# Autodesk Inventor assembly: Box Arm
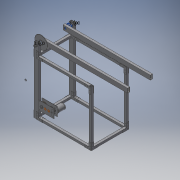
[picture p0: Inventor's stored thumbnail of the model, 180x180]
Saved by Autodesk Inventor 2018 (Build 220112000, 112)
## iProperties
Created: 2019-01-16
Part Number: Box Arm
Document SubType Name: Assembly
Designer: Gabriel
Author: Gabriel
## Documents named in this file (27)
- C:\Users\S-2513398\Downloads\2019CAD-master\2019CAD-master\Drivebase Box Arm\Box Arm.iam
- C:\Users\S-2513398\Downloads\2019CAD-master\2019CAD-master\Drivebase Box Arm\30in 1x1 Beam.ipt
- C:\Users\S-2513398\Downloads\2019CAD-master\2019CAD-master\Drivebase Box Arm\25in 1x1 Beam.ipt
- C:\Users\S-2513398\Downloads\2019CAD-master\2019CAD-master\Drivebase Box Arm\17in 1x1 Beam.ipt
- C:\Users\S-2513398\Downloads\2019CAD-master\2019CAD-master\Drivebase Box Arm\23in 1x1 Beam.ipt
- C:\Users\S-2513398\Downloads\2019CAD-master\2019CAD-master\Drivebase Box Arm\L gusset.ipt
- C:\Users\S-2513398\Downloads\2019CAD-master\2019CAD-master\Drivebase Box Arm\34.48in Arm Bea.ipt
- C:\Users\S-2513398\Downloads\2019CAD-master\2019CAD-master\Drivebase Box Arm\0_500_ID_x_1_125_OD_x_0_313_WD_Flanged_Bearing_217-2731.ipt
- C:\Users\S-2513398\Downloads\2019CAD-master\2019CAD-master\Drivebase Box Arm\_72t_Aluminum_Plate_Sprocket_25_Chain_1-1_8_Bearing_Bore_217-2627.ipt
- C:\Users\S-2513398\Downloads\2019CAD-master\2019CAD-master\Drivebase Box Arm\Hex Hub.ipt
- C:\Users\S-2513398\Downloads\2019CAD-master\2019CAD-master\Drivebase Box Arm\0.5in Hex Shaft.ipt
- C:\Users\S-2513398\Downloads\2019CAD-master\2019CAD-master\Drivebase Box Arm\1_2_Acetal_Spacer_-_1_2_Hex_217-3261.ipt
- C:\Users\S-2513398\Downloads\2019CAD-master\2019CAD-master\Drivebase Box Arm\am-0150 Toughbox Large Output Gear.ipt
- C:\Users\S-2513398\Downloads\2019CAD-master\2019CAD-master\Drivebase Box Arm\Mini_CIM_Motor_217-3371.ipt
- C:\Users\S-2513398\Downloads\2019CAD-master\2019CAD-master\Drivebase Box Arm\ARm Gearbox Plate.ipt
- C:\Users\S-2513398\Downloads\2019CAD-master\2019CAD-master\Drivebase Box Arm\1_16_Acetal_Spacer_-_1_2_Hex_217-3257.ipt
- C:\Users\S-2513398\Downloads\2019CAD-master\2019CAD-master\Drivebase Box Arm\3_8in Hex Shaft.ipt
- C:\Users\S-2513398\Downloads\2019CAD-master\2019CAD-master\Drivebase Box Arm\10T_Steel_Spur_Gear_20_DP_12T_Center_Distance_CIM_Motor_217-6334.ipt
- C:\Users\S-2513398\Downloads\2019CAD-master\2019CAD-master\Drivebase Box Arm\am-0143 50 Tooth 20 dp Aluminum Gear 375 Hex.ipt
- C:\Users\S-2513398\Downloads\2019CAD-master\2019CAD-master\Drivebase Box Arm\am-0151 14T 20dp 375hex.ipt
- C:\Users\S-2513398\Downloads\2019CAD-master\2019CAD-master\Drivebase Box Arm\1_16_Acetal_Spacer_-_3_8_Hex_217-3258.ipt
- C:\Users\S-2513398\Downloads\2019CAD-master\2019CAD-master\Drivebase Box Arm\40t_Aluminum_Spur_Gear_20_DP_3_8_Hex_Bore_217-2707.ipt
- C:\Users\S-2513398\Downloads\2019CAD-master\2019CAD-master\Drivebase Box Arm\am-0028 00.375'' id Flanged, Shielded Ball Bearing (FR6ZZ).ipt
- C:\Users\S-2513398\Downloads\2019CAD-master\2019CAD-master\Drivebase Box Arm\92196A271_18-8 STAINLESS STEEL SOCKET HEAD CAP SCREW.ipt
- C:\Users\S-2513398\Downloads\2019CAD-master\2019CAD-master\Drivebase Box Arm\am-3621 - S25-18HA-500H.ipt
- C:\Users\S-2513398\Downloads\2019CAD-master\2019CAD-master\Drivebase Box Arm\Clamping_Shaft_Collar_-_1_2_Hex_ID_217-2737.ipt
- C:\Users\S-2513398\Downloads\#10 Washer.ipt
## Components (89 placed, 26 different names)
1. 30in 1x1 Beam:1 — Mate:13, Mate:14, Mate:37, Mate:38, Mate:74, Mate:75, Mate:83, Mate:84, Mate:98, Mate:99, Mate:101, Mate:102, Mate:103, Mate:104
2. 30in 1x1 Beam:2 — Mate:11, Mate:12, Mate:39, Mate:40, Mate:73, Mate:76, Mate:86, Mate:87, Mate:95, Mate:96, Mate:105, Mate:106, Mate:107, Mate:108, Mate:441, Mate:442
3. 25in 1x1 Beam:1 — Mate:57, Mate:58, Mate:59, Mate:60, Mate:65, Mate:66, Mate:90, Mate:91
4. 25in 1x1 Beam:2 — Mate:61, Mate:62, Mate:63, Mate:64, Mate:67, Mate:68, Mate:93, Mate:94
5. 25in 1x1 Beam:3 — Mate:29, Mate:30, Mate:53, Mate:54, Mate:97, Mate:443
6. 25in 1x1 Beam:4 — Mate:31, Mate:32, Mate:55, Mate:56, Mate:100
7. 17in 1x1 Beam:1 — Mate:69, Mate:70, Mate:71, Mate:72
8. 17in 1x1 Beam:2 — Mate:21, Mate:22, Mate:23, Mate:24
9. 23in 1x1 Beam:1 — Mate:43, Mate:44, Mate:49, Mate:50, Mate:88, Mate:92
10. 23in 1x1 Beam:2 — Mate:47, Mate:48, Mate:51, Mate:52, Mate:85, Mate:89
11. L gusset:1 — Mate:53, Mate:54, Mate:63, Mate:64
12. L gusset:4 — Mate:49, Mate:50, Mate:61, Mate:62
13. L gusset:5 — Mate:51, Mate:52, Mate:57, Mate:58
14. L gusset:7 — Mate:11, Mate:12, Mate:23, Mate:24
15. L gusset:9 — Mate:13, Mate:14, Mate:21, Mate:22
16. L gusset:11 — Mate:31, Mate:32, Mate:74, Mate:75
17. L gusset:12 — Mate:29, Mate:30, Mate:73, Mate:76
18. L gusset:13 — Mate:43, Mate:44
19. L gusset:14 — Mate:47, Mate:48
20. L gusset:15 — Mate:39, Mate:40, Mate:77, Mate:80
21. L gusset:16 — Mate:37, Mate:38, Mate:78, Mate:79
22. L gusset:17 — Mate:55, Mate:56, Mate:59, Mate:60
23. L gusset:18 — Mate:67, Mate:68, Mate:69, Mate:70
24. L gusset:19 — Mate:65, Mate:66, Mate:71, Mate:72
25. 17in 1x1 Beam:3 — Mate:77, Mate:78, Mate:79, Mate:80
26. 34.48in Arm Bea:2 — Mate:109, Mate:110
27. 0_500_ID_x_1_125_OD_x_0_313_WD_Flanged_Bearing_217-2731:1 — Mate:103, Mate:104, Mate:139, Mate:140, Mate:149
28. 0_500_ID_x_1_125_OD_x_0_313_WD_Flanged_Bearing_217-2731:2 — Mate:107, Mate:108, Mate:126, Mate:152
29. 0_500_ID_x_1_125_OD_x_0_313_WD_Flanged_Bearing_217-2731:5 — Mate:101, Mate:102, Mate:143
30. 0_500_ID_x_1_125_OD_x_0_313_WD_Flanged_Bearing_217-2731:8 — Mate:105, Mate:106, Mate:446, Mate:447
31. L gusset:20 — Mate:92, Mate:93, Mate:94
32. L gusset:21 — Mate:89, Mate:90, Mate:91
33. L gusset:22 — Mate:98, Mate:99, Mate:100
34. L gusset:23 — Mate:95, Mate:96, Mate:97
35. L gusset:24 — Mate:83, Mate:84, Mate:85
36. L gusset:25 — Mate:86, Mate:87, Mate:88
37. _72t_Aluminum_Plate_Sprocket_25_Chain_1-1_8_Bearing_Bore_217-2627:2 — Mate:120, Mate:121, Mate:138, Flush:4
38. Hex Hub:2 — Mate:109, Mate:110, Mate:111, Mate:112, Mate:113
39. Hex Hub:3 — Mate:120, Mate:121, Mate:138, Mate:444, Mate:445
40. 1_2_Acetal_Spacer_-_1_2_Hex_217-3261:1 — Mate:126, Mate:406
41. 1_2_Acetal_Spacer_-_1_2_Hex_217-3261:3 — Mate:111, Mate:112, Mate:113
42. 34.48in Arm Bea:3 — Mate:128
43. Hex Hub:4 — Mate:136, Mate:139, Mate:140
44. Hex Hub:5 — Mate:128, Mate:133
45. 1_2_Acetal_Spacer_-_1_2_Hex_217-3261:7 — Mate:143, Mate:403
46. 1_2_Acetal_Spacer_-_1_2_Hex_217-3261:8 — Mate:133, Mate:136
47. 1_2_Acetal_Spacer_-_1_2_Hex_217-3261:9 — Mate:149
48. 1_2_Acetal_Spacer_-_1_2_Hex_217-3261:10 — Mate:152
49. 0.5in Hex Shaft:5 — Mate:345, Mate:346, Mate:347, Mate:348, Mate:349, Mate:350, Mate:351, Mate:386, Mate:387, Mate:389, Mate:390, Mate:395, Mate:396, Mate:398, Mate:399, Rotation:1, Mate:437, Mate:438, Flush:3
50. Mini_CIM_Motor_217-3371:5 — Mate:431, Mate:432, Mate:433, Mate:434, Mate:435, Mate:436
51. am-0150 Toughbox Large Output Gear:8 — Mate:345, Mate:346, Mate:347, Mate:352
52. 1_16_Acetal_Spacer_-_1_2_Hex_217-3257:4 — Mate:348, Mate:349, Mate:352, Mate:353
53. 1_16_Acetal_Spacer_-_1_2_Hex_217-3257:6 — Mate:350, Mate:351, Mate:353, Mate:354
54. 3_8in Hex Shaft:5 — Mate:313, Mate:314, Mate:315, Mate:316, Mate:317, Mate:318, Mate:321, Mate:322, Mate:357, Mate:358, Mate:411, Flush:2, Mate:425, Rotation:2
55. am-0151 14T 20dp 375hex:1 — Mate:325, Mate:326, Mate:331, Mate:335
56. am-0151 14T 20dp 375hex:3 — Mate:315, Mate:316, Mate:320, Mate:359
57. am-0143 50 Tooth 20 dp Aluminum Gear 375 Hex:5 — Mate:327, Mate:328, Mate:332, Mate:339
58. 10T_Steel_Spur_Gear_20_DP_12T_Center_Distance_CIM_Motor_217-6334:6 — Mate:434, Mate:435, Mate:436
59. 1_16_Acetal_Spacer_-_3_8_Hex_217-3258:2 — Mate:337, Mate:338, Mate:339
60. 1_16_Acetal_Spacer_-_3_8_Hex_217-3258:3 — Mate:333, Mate:334, Mate:335, Mate:422
61. 1_16_Acetal_Spacer_-_3_8_Hex_217-3258:5 — Mate:321, Mate:322, Mate:323, Mate:423
62. 1_16_Acetal_Spacer_-_3_8_Hex_217-3258:6 — Mate:317, Mate:318, Mate:319, Mate:320
63. 40t_Aluminum_Spur_Gear_20_DP_3_8_Hex_Bore_217-2707:1 — Mate:313, Mate:314, Mate:319, Mate:323
64. 3_8in Hex Shaft:10 — Mate:325, Mate:326, Mate:327, Mate:328, Mate:329, Mate:330, Mate:333, Mate:334, Mate:337, Mate:338, Mate:412, Flush:1, Mate:424, Mate:426, Rotation:3
65. ARm Gearbox Plate:5 — Mate:341, Mate:344, Mate:413, Mate:414, Mate:415, Mate:416, Mate:441, Mate:442, Mate:443
66. ARm Gearbox Plate:6 — Mate:342, Mate:343, Mate:360, Mate:361, Mate:362, Mate:363, Mate:407, Mate:408, Mate:409, Mate:410, Mate:419, Mate:421, Rotation:1
67. 1_16_Acetal_Spacer_-_3_8_Hex_217-3258:8 — Mate:357, Mate:358, Mate:359
68. 1_16_Acetal_Spacer_-_3_8_Hex_217-3258:10 — Mate:329, Mate:330, Mate:331, Mate:332
69. 0_500_ID_x_1_125_OD_x_0_313_WD_Flanged_Bearing_217-2731:9 — Mate:341, Mate:344, Mate:439
70. 0_500_ID_x_1_125_OD_x_0_313_WD_Flanged_Bearing_217-2731:10 — Mate:342, Mate:343, Mate:354
71. 92196A271_18-8 STAINLESS STEEL SOCKET HEAD CAP SCREW:1 — Mate:361, Mate:363, Mate:420, Mate:429, Mate:431
72. 92196A271_18-8 STAINLESS STEEL SOCKET HEAD CAP SCREW:2 — Mate:360, Mate:362, Mate:417, Mate:427, Mate:432
73. am-0028 00.375'' id Flanged, Shielded Ball Bearing (FR6ZZ):3 — Mate:414, Mate:416, Mate:425, Rotation:2
74. am-0028 00.375'' id Flanged, Shielded Ball Bearing (FR6ZZ):4 — Mate:413, Mate:415, Mate:424, Mate:426, Rotation:3
75. am-3621 - S25-18HA-500H:1 — Mate:386, Mate:387, Flush:4
76. 1_2_Acetal_Spacer_-_1_2_Hex_217-3261:11 — Mate:389, Mate:390, Mate:397
77. Clamping_Shaft_Collar_-_1_2_Hex_ID_217-2737:1 — Mate:395, Mate:396, Mate:397, Flush:3
78. Clamping_Shaft_Collar_-_1_2_Hex_ID_217-2737:2 — Mate:398, Mate:399, Mate:440
79. Clamping_Shaft_Collar_-_1_2_Hex_ID_217-2737:5 — Mate:406
80. Clamping_Shaft_Collar_-_1_2_Hex_ID_217-2737:6 — Mate:403
81. am-0028 00.375'' id Flanged, Shielded Ball Bearing (FR6ZZ):5 — Mate:409, Mate:410, Mate:411, Flush:2, Mate:423
82. am-0028 00.375'' id Flanged, Shielded Ball Bearing (FR6ZZ):6 — Mate:407, Mate:408, Mate:412, Flush:1, Mate:422
83. #10 Washer:1 — Mate:417, Mate:419, Mate:428
84. #10 Washer:2 — Mate:420, Mate:421, Mate:430
85. #10 Washer:3 — Mate:427, Mate:428, Mate:433
86. #10 Washer:4 — Mate:429, Mate:430
87. 1_16_Acetal_Spacer_-_1_2_Hex_217-3257:9 — Mate:437, Mate:438, Mate:439, Mate:440
88. 1_16_Acetal_Spacer_-_1_2_Hex_217-3257:10
89. 1_2_Acetal_Spacer_-_1_2_Hex_217-3261:12 — Mate:444, Mate:445, Mate:446, Mate:447
## Relationships (199: Mate 192, Flush 4, RelateRotation 3)
- Mate:11: 30in 1x1 Beam:2 ↔ L gusset:7
- Mate:12: 30in 1x1 Beam:2 ↔ L gusset:7
- Mate:13: 30in 1x1 Beam:1 ↔ L gusset:9
- Mate:14: 30in 1x1 Beam:1 ↔ L gusset:9
- Mate:21: 17in 1x1 Beam:2 ↔ L gusset:9
- Mate:22: 17in 1x1 Beam:2 ↔ L gusset:9
- Mate:23: 17in 1x1 Beam:2 ↔ L gusset:7
- Mate:24: 17in 1x1 Beam:2 ↔ L gusset:7
- Mate:29: 25in 1x1 Beam:3 ↔ L gusset:12
- Mate:30: 25in 1x1 Beam:3 ↔ L gusset:12
- Mate:31: 25in 1x1 Beam:4 ↔ L gusset:11
- Mate:32: 25in 1x1 Beam:4 ↔ L gusset:11
- Mate:37: 30in 1x1 Beam:1 ↔ L gusset:16
- Mate:38: 30in 1x1 Beam:1 ↔ L gusset:16
- Mate:39: 30in 1x1 Beam:2 ↔ L gusset:15
- Mate:40: 30in 1x1 Beam:2 ↔ L gusset:15
- Mate:43: 23in 1x1 Beam:1 ↔ L gusset:13
- Mate:44: 23in 1x1 Beam:1 ↔ L gusset:13
- Mate:47: 23in 1x1 Beam:2 ↔ L gusset:14
- Mate:48: 23in 1x1 Beam:2 ↔ L gusset:14
- Mate:49: 23in 1x1 Beam:1 ↔ L gusset:4
- Mate:50: 23in 1x1 Beam:1 ↔ L gusset:4
- Mate:51: 23in 1x1 Beam:2 ↔ L gusset:5
- Mate:52: 23in 1x1 Beam:2 ↔ L gusset:5
- Mate:53: 25in 1x1 Beam:3 ↔ L gusset:1
- Mate:54: 25in 1x1 Beam:3 ↔ L gusset:1
- Mate:55: 25in 1x1 Beam:4 ↔ L gusset:17
- Mate:56: 25in 1x1 Beam:4 ↔ L gusset:17
- Mate:57: 25in 1x1 Beam:1 ↔ L gusset:5
- Mate:58: 25in 1x1 Beam:1 ↔ L gusset:5
- Mate:59: 25in 1x1 Beam:1 ↔ L gusset:17
- Mate:60: 25in 1x1 Beam:1 ↔ L gusset:17
- Mate:61: 25in 1x1 Beam:2 ↔ L gusset:4
- Mate:62: 25in 1x1 Beam:2 ↔ L gusset:4
- Mate:63: 25in 1x1 Beam:2 ↔ L gusset:1
- Mate:64: 25in 1x1 Beam:2 ↔ L gusset:1
- Mate:65: 25in 1x1 Beam:1 ↔ L gusset:19
- Mate:66: 25in 1x1 Beam:1 ↔ L gusset:19
- Mate:67: 25in 1x1 Beam:2 ↔ L gusset:18
- Mate:68: 25in 1x1 Beam:2 ↔ L gusset:18
- Mate:69: 17in 1x1 Beam:1 ↔ L gusset:18
- Mate:70: 17in 1x1 Beam:1 ↔ L gusset:18
- Mate:71: 17in 1x1 Beam:1 ↔ L gusset:19
- Mate:72: 17in 1x1 Beam:1 ↔ L gusset:19
- Mate:73: 30in 1x1 Beam:2 ↔ L gusset:12
- Mate:74: 30in 1x1 Beam:1 ↔ L gusset:11
- Mate:75: 30in 1x1 Beam:1 ↔ L gusset:11
- Mate:76: 30in 1x1 Beam:2 ↔ L gusset:12
- Mate:77: L gusset:15 ↔ 17in 1x1 Beam:3
- Mate:78: L gusset:16 ↔ 17in 1x1 Beam:3
- Mate:79: L gusset:16 ↔ 17in 1x1 Beam:3
- Mate:80: L gusset:15 ↔ 17in 1x1 Beam:3
- Mate:83: 30in 1x1 Beam:1 ↔ L gusset:24
- Mate:84: 30in 1x1 Beam:1 ↔ L gusset:24
- Mate:85: 23in 1x1 Beam:2 ↔ L gusset:24
- Mate:86: 30in 1x1 Beam:2 ↔ L gusset:25
- Mate:87: 30in 1x1 Beam:2 ↔ L gusset:25
- Mate:88: 23in 1x1 Beam:1 ↔ L gusset:25
- Mate:89: 23in 1x1 Beam:2 ↔ L gusset:21
- Mate:90: 25in 1x1 Beam:1 ↔ L gusset:21
- Mate:91: 25in 1x1 Beam:1 ↔ L gusset:21
- Mate:92: 23in 1x1 Beam:1 ↔ L gusset:20
- Mate:93: 25in 1x1 Beam:2 ↔ L gusset:20
- Mate:94: 25in 1x1 Beam:2 ↔ L gusset:20
- Mate:95: 30in 1x1 Beam:2 ↔ L gusset:23
- Mate:96: 30in 1x1 Beam:2 ↔ L gusset:23
- Mate:97: 25in 1x1 Beam:3 ↔ L gusset:23
- Mate:98: 30in 1x1 Beam:1 ↔ L gusset:22
- Mate:99: 30in 1x1 Beam:1 ↔ L gusset:22
- Mate:100: 25in 1x1 Beam:4 ↔ L gusset:22
- Mate:101: 30in 1x1 Beam:1 ↔ 0_500_ID_x_1_125_OD_x_0_313_WD_Flanged_Bearing_217-2731:5
- Mate:102: 30in 1x1 Beam:1 ↔ 0_500_ID_x_1_125_OD_x_0_313_WD_Flanged_Bearing_217-2731:5
- Mate:103: 30in 1x1 Beam:1 ↔ 0_500_ID_x_1_125_OD_x_0_313_WD_Flanged_Bearing_217-2731:1
- Mate:104: 30in 1x1 Beam:1 ↔ 0_500_ID_x_1_125_OD_x_0_313_WD_Flanged_Bearing_217-2731:1
- Mate:105: 30in 1x1 Beam:2 ↔ 0_500_ID_x_1_125_OD_x_0_313_WD_Flanged_Bearing_217-2731:8
- Mate:106: 30in 1x1 Beam:2 ↔ 0_500_ID_x_1_125_OD_x_0_313_WD_Flanged_Bearing_217-2731:8
- Mate:107: 30in 1x1 Beam:2 ↔ 0_500_ID_x_1_125_OD_x_0_313_WD_Flanged_Bearing_217-2731:2
- Mate:108: 30in 1x1 Beam:2 ↔ 0_500_ID_x_1_125_OD_x_0_313_WD_Flanged_Bearing_217-2731:2
- Mate:109: 34.48in Arm Bea:2 ↔ Hex Hub:2
- Mate:110: 34.48in Arm Bea:2 ↔ Hex Hub:2
- Mate:111: Hex Hub:2 ↔ 1_2_Acetal_Spacer_-_1_2_Hex_217-3261:3
- Mate:112: Hex Hub:2 ↔ 1_2_Acetal_Spacer_-_1_2_Hex_217-3261:3
- Mate:113: Hex Hub:2 ↔ 1_2_Acetal_Spacer_-_1_2_Hex_217-3261:3
- Mate:120: _72t_Aluminum_Plate_Sprocket_25_Chain_1-1_8_Bearing_Bore_217-2627:2 ↔ Hex Hub:3
- Mate:121: _72t_Aluminum_Plate_Sprocket_25_Chain_1-1_8_Bearing_Bore_217-2627:2 ↔ Hex Hub:3
- Mate:126: 0_500_ID_x_1_125_OD_x_0_313_WD_Flanged_Bearing_217-2731:2 ↔ 1_2_Acetal_Spacer_-_1_2_Hex_217-3261:1
- Mate:128: 34.48in Arm Bea:3 ↔ Hex Hub:5
- Mate:133: Hex Hub:5 ↔ 1_2_Acetal_Spacer_-_1_2_Hex_217-3261:8
- Mate:136: Hex Hub:4 ↔ 1_2_Acetal_Spacer_-_1_2_Hex_217-3261:8
- Mate:138: _72t_Aluminum_Plate_Sprocket_25_Chain_1-1_8_Bearing_Bore_217-2627:2 ↔ Hex Hub:3
- Mate:139: 0_500_ID_x_1_125_OD_x_0_313_WD_Flanged_Bearing_217-2731:1 ↔ Hex Hub:4
- Mate:140: 0_500_ID_x_1_125_OD_x_0_313_WD_Flanged_Bearing_217-2731:1 ↔ Hex Hub:4
- Mate:143: 0_500_ID_x_1_125_OD_x_0_313_WD_Flanged_Bearing_217-2731:5 ↔ 1_2_Acetal_Spacer_-_1_2_Hex_217-3261:7
- Mate:149: 0_500_ID_x_1_125_OD_x_0_313_WD_Flanged_Bearing_217-2731:1 ↔ 1_2_Acetal_Spacer_-_1_2_Hex_217-3261:9
- Mate:152: 0_500_ID_x_1_125_OD_x_0_313_WD_Flanged_Bearing_217-2731:2 ↔ 1_2_Acetal_Spacer_-_1_2_Hex_217-3261:10
- Mate:313: 3_8in Hex Shaft:5 ↔ 40t_Aluminum_Spur_Gear_20_DP_3_8_Hex_Bore_217-2707:1
- Mate:314: 3_8in Hex Shaft:5 ↔ 40t_Aluminum_Spur_Gear_20_DP_3_8_Hex_Bore_217-2707:1
- Mate:315: 3_8in Hex Shaft:5 ↔ am-0151 14T 20dp 375hex:3
- Mate:316: 3_8in Hex Shaft:5 ↔ am-0151 14T 20dp 375hex:3
- Mate:317: 3_8in Hex Shaft:5 ↔ 1_16_Acetal_Spacer_-_3_8_Hex_217-3258:6
- Mate:318: 3_8in Hex Shaft:5 ↔ 1_16_Acetal_Spacer_-_3_8_Hex_217-3258:6
- Mate:319: 1_16_Acetal_Spacer_-_3_8_Hex_217-3258:6 ↔ 40t_Aluminum_Spur_Gear_20_DP_3_8_Hex_Bore_217-2707:1
- Mate:320: am-0151 14T 20dp 375hex:3 ↔ 1_16_Acetal_Spacer_-_3_8_Hex_217-3258:6
- Mate:321: 3_8in Hex Shaft:5 ↔ 1_16_Acetal_Spacer_-_3_8_Hex_217-3258:5
- Mate:322: 3_8in Hex Shaft:5 ↔ 1_16_Acetal_Spacer_-_3_8_Hex_217-3258:5
- Mate:323: 1_16_Acetal_Spacer_-_3_8_Hex_217-3258:5 ↔ 40t_Aluminum_Spur_Gear_20_DP_3_8_Hex_Bore_217-2707:1
- Mate:325: am-0151 14T 20dp 375hex:1 ↔ 3_8in Hex Shaft:10
- Mate:326: am-0151 14T 20dp 375hex:1 ↔ 3_8in Hex Shaft:10
- Mate:327: am-0143 50 Tooth 20 dp Aluminum Gear 375 Hex:5 ↔ 3_8in Hex Shaft:10
- Mate:328: am-0143 50 Tooth 20 dp Aluminum Gear 375 Hex:5 ↔ 3_8in Hex Shaft:10
- Mate:329: 3_8in Hex Shaft:10 ↔ 1_16_Acetal_Spacer_-_3_8_Hex_217-3258:10
- Mate:330: 3_8in Hex Shaft:10 ↔ 1_16_Acetal_Spacer_-_3_8_Hex_217-3258:10
- Mate:331: am-0151 14T 20dp 375hex:1 ↔ 1_16_Acetal_Spacer_-_3_8_Hex_217-3258:10
- Mate:332: am-0143 50 Tooth 20 dp Aluminum Gear 375 Hex:5 ↔ 1_16_Acetal_Spacer_-_3_8_Hex_217-3258:10
- Mate:333: 1_16_Acetal_Spacer_-_3_8_Hex_217-3258:3 ↔ 3_8in Hex Shaft:10
- Mate:334: 1_16_Acetal_Spacer_-_3_8_Hex_217-3258:3 ↔ 3_8in Hex Shaft:10
- Mate:335: am-0151 14T 20dp 375hex:1 ↔ 1_16_Acetal_Spacer_-_3_8_Hex_217-3258:3
- Mate:337: 1_16_Acetal_Spacer_-_3_8_Hex_217-3258:2 ↔ 3_8in Hex Shaft:10
- Mate:338: 1_16_Acetal_Spacer_-_3_8_Hex_217-3258:2 ↔ 3_8in Hex Shaft:10
- Mate:339: am-0143 50 Tooth 20 dp Aluminum Gear 375 Hex:5 ↔ 1_16_Acetal_Spacer_-_3_8_Hex_217-3258:2
- Mate:341: ARm Gearbox Plate:5 ↔ 0_500_ID_x_1_125_OD_x_0_313_WD_Flanged_Bearing_217-2731:9
- Mate:342: ARm Gearbox Plate:6 ↔ 0_500_ID_x_1_125_OD_x_0_313_WD_Flanged_Bearing_217-2731:10
- Mate:343: ARm Gearbox Plate:6 ↔ 0_500_ID_x_1_125_OD_x_0_313_WD_Flanged_Bearing_217-2731:10
- Mate:344: ARm Gearbox Plate:5 ↔ 0_500_ID_x_1_125_OD_x_0_313_WD_Flanged_Bearing_217-2731:9
- Mate:345: 0.5in Hex Shaft:5 ↔ am-0150 Toughbox Large Output Gear:8
- Mate:346: 0.5in Hex Shaft:5 ↔ am-0150 Toughbox Large Output Gear:8
- Mate:347: 0.5in Hex Shaft:5 ↔ am-0150 Toughbox Large Output Gear:8
- Mate:348: 0.5in Hex Shaft:5 ↔ 1_16_Acetal_Spacer_-_1_2_Hex_217-3257:4
- Mate:349: 0.5in Hex Shaft:5 ↔ 1_16_Acetal_Spacer_-_1_2_Hex_217-3257:4
- Mate:350: 0.5in Hex Shaft:5 ↔ 1_16_Acetal_Spacer_-_1_2_Hex_217-3257:6
- Mate:351: 0.5in Hex Shaft:5 ↔ 1_16_Acetal_Spacer_-_1_2_Hex_217-3257:6
- Mate:352: am-0150 Toughbox Large Output Gear:8 ↔ 1_16_Acetal_Spacer_-_1_2_Hex_217-3257:4
- Mate:353: 1_16_Acetal_Spacer_-_1_2_Hex_217-3257:4 ↔ 1_16_Acetal_Spacer_-_1_2_Hex_217-3257:6
- Mate:354: 1_16_Acetal_Spacer_-_1_2_Hex_217-3257:6 ↔ 0_500_ID_x_1_125_OD_x_0_313_WD_Flanged_Bearing_217-2731:10
- Mate:357: 3_8in Hex Shaft:5 ↔ 1_16_Acetal_Spacer_-_3_8_Hex_217-3258:8
- Mate:358: 3_8in Hex Shaft:5 ↔ 1_16_Acetal_Spacer_-_3_8_Hex_217-3258:8
- Mate:359: am-0151 14T 20dp 375hex:3 ↔ 1_16_Acetal_Spacer_-_3_8_Hex_217-3258:8
- Mate:360: ARm Gearbox Plate:6 ↔ 92196A271_18-8 STAINLESS STEEL SOCKET HEAD CAP SCREW:2
- Mate:361: ARm Gearbox Plate:6 ↔ 92196A271_18-8 STAINLESS STEEL SOCKET HEAD CAP SCREW:1
- Mate:362: ARm Gearbox Plate:6 ↔ 92196A271_18-8 STAINLESS STEEL SOCKET HEAD CAP SCREW:2
- Mate:363: ARm Gearbox Plate:6 ↔ 92196A271_18-8 STAINLESS STEEL SOCKET HEAD CAP SCREW:1
- Mate:386: 0.5in Hex Shaft:5 ↔ am-3621 - S25-18HA-500H:1
- Mate:387: 0.5in Hex Shaft:5 ↔ am-3621 - S25-18HA-500H:1
- Mate:389: 0.5in Hex Shaft:5 ↔ 1_2_Acetal_Spacer_-_1_2_Hex_217-3261:11
- Mate:390: 0.5in Hex Shaft:5 ↔ 1_2_Acetal_Spacer_-_1_2_Hex_217-3261:11
- Mate:395: 0.5in Hex Shaft:5 ↔ Clamping_Shaft_Collar_-_1_2_Hex_ID_217-2737:1
- Mate:396: 0.5in Hex Shaft:5 ↔ Clamping_Shaft_Collar_-_1_2_Hex_ID_217-2737:1
- Mate:397: 1_2_Acetal_Spacer_-_1_2_Hex_217-3261:11 ↔ Clamping_Shaft_Collar_-_1_2_Hex_ID_217-2737:1
- Mate:398: 0.5in Hex Shaft:5 ↔ Clamping_Shaft_Collar_-_1_2_Hex_ID_217-2737:2
- Mate:399: 0.5in Hex Shaft:5 ↔ Clamping_Shaft_Collar_-_1_2_Hex_ID_217-2737:2
- Mate:403: 1_2_Acetal_Spacer_-_1_2_Hex_217-3261:7 ↔ Clamping_Shaft_Collar_-_1_2_Hex_ID_217-2737:6
- Mate:406: 1_2_Acetal_Spacer_-_1_2_Hex_217-3261:1 ↔ Clamping_Shaft_Collar_-_1_2_Hex_ID_217-2737:5
- Mate:407: ARm Gearbox Plate:6 ↔ am-0028 00.375'' id Flanged, Shielded Ball Bearing (FR6ZZ):6
- Mate:408: ARm Gearbox Plate:6 ↔ am-0028 00.375'' id Flanged, Shielded Ball Bearing (FR6ZZ):6
- Mate:409: ARm Gearbox Plate:6 ↔ am-0028 00.375'' id Flanged, Shielded Ball Bearing (FR6ZZ):5
- Mate:410: ARm Gearbox Plate:6 ↔ am-0028 00.375'' id Flanged, Shielded Ball Bearing (FR6ZZ):5
- Mate:411: 3_8in Hex Shaft:5 ↔ am-0028 00.375'' id Flanged, Shielded Ball Bearing (FR6ZZ):5
- Mate:412: 3_8in Hex Shaft:10 ↔ am-0028 00.375'' id Flanged, Shielded Ball Bearing (FR6ZZ):6
- Mate:413: ARm Gearbox Plate:5 ↔ am-0028 00.375'' id Flanged, Shielded Ball Bearing (FR6ZZ):4
- Mate:414: ARm Gearbox Plate:5 ↔ am-0028 00.375'' id Flanged, Shielded Ball Bearing (FR6ZZ):3
- Mate:415: ARm Gearbox Plate:5 ↔ am-0028 00.375'' id Flanged, Shielded Ball Bearing (FR6ZZ):4
- Mate:416: ARm Gearbox Plate:5 ↔ am-0028 00.375'' id Flanged, Shielded Ball Bearing (FR6ZZ):3
- Mate:417: 92196A271_18-8 STAINLESS STEEL SOCKET HEAD CAP SCREW:2 ↔ #10 Washer:1
- Mate:419: ARm Gearbox Plate:6 ↔ #10 Washer:1
- Mate:420: 92196A271_18-8 STAINLESS STEEL SOCKET HEAD CAP SCREW:1 ↔ #10 Washer:2
- Mate:421: ARm Gearbox Plate:6 ↔ #10 Washer:2
- Flush:1: 3_8in Hex Shaft:10 ↔ am-0028 00.375'' id Flanged, Shielded Ball Bearing (FR6ZZ):6
- Flush:2: 3_8in Hex Shaft:5 ↔ am-0028 00.375'' id Flanged, Shielded Ball Bearing (FR6ZZ):5
- Rotation:1 [RelateRotation] (1 ul): 0.5in Hex Shaft:5 ↔ ARm Gearbox Plate:6
- Mate:422: 1_16_Acetal_Spacer_-_3_8_Hex_217-3258:3 ↔ am-0028 00.375'' id Flanged, Shielded Ball Bearing (FR6ZZ):6
- Mate:423: 1_16_Acetal_Spacer_-_3_8_Hex_217-3258:5 ↔ am-0028 00.375'' id Flanged, Shielded Ball Bearing (FR6ZZ):5
- Mate:424: 3_8in Hex Shaft:10 ↔ am-0028 00.375'' id Flanged, Shielded Ball Bearing (FR6ZZ):4
- Mate:425: 3_8in Hex Shaft:5 ↔ am-0028 00.375'' id Flanged, Shielded Ball Bearing (FR6ZZ):3
- Mate:426: 3_8in Hex Shaft:10 ↔ am-0028 00.375'' id Flanged, Shielded Ball Bearing (FR6ZZ):4
- Rotation:2 [RelateRotation] (1 ul): 3_8in Hex Shaft:5 ↔ am-0028 00.375'' id Flanged, Shielded Ball Bearing (FR6ZZ):3
- Rotation:3 [RelateRotation] (1 ul): 3_8in Hex Shaft:10 ↔ am-0028 00.375'' id Flanged, Shielded Ball Bearing (FR6ZZ):4
- Mate:427: 92196A271_18-8 STAINLESS STEEL SOCKET HEAD CAP SCREW:2 ↔ #10 Washer:3
- Mate:428: #10 Washer:1 ↔ #10 Washer:3
- Mate:429: 92196A271_18-8 STAINLESS STEEL SOCKET HEAD CAP SCREW:1 ↔ #10 Washer:4
- Mate:430: #10 Washer:2 ↔ #10 Washer:4
- Mate:431: Mini_CIM_Motor_217-3371:5 ↔ 92196A271_18-8 STAINLESS STEEL SOCKET HEAD CAP SCREW:1
- Mate:432: Mini_CIM_Motor_217-3371:5 ↔ 92196A271_18-8 STAINLESS STEEL SOCKET HEAD CAP SCREW:2
- Mate:433: Mini_CIM_Motor_217-3371:5 ↔ #10 Washer:3
- Mate:434: Mini_CIM_Motor_217-3371:5 ↔ 10T_Steel_Spur_Gear_20_DP_12T_Center_Distance_CIM_Motor_217-6334:6
- Mate:435: Mini_CIM_Motor_217-3371:5 ↔ 10T_Steel_Spur_Gear_20_DP_12T_Center_Distance_CIM_Motor_217-6334:6
- Mate:436: Mini_CIM_Motor_217-3371:5 ↔ 10T_Steel_Spur_Gear_20_DP_12T_Center_Distance_CIM_Motor_217-6334:6
- Mate:437: 0.5in Hex Shaft:5 ↔ 1_16_Acetal_Spacer_-_1_2_Hex_217-3257:9
- Mate:438: 0.5in Hex Shaft:5 ↔ 1_16_Acetal_Spacer_-_1_2_Hex_217-3257:9
- Mate:439: 0_500_ID_x_1_125_OD_x_0_313_WD_Flanged_Bearing_217-2731:9 ↔ 1_16_Acetal_Spacer_-_1_2_Hex_217-3257:9
- Mate:440: Clamping_Shaft_Collar_-_1_2_Hex_ID_217-2737:2 ↔ 1_16_Acetal_Spacer_-_1_2_Hex_217-3257:9
- Flush:3: 0.5in Hex Shaft:5 ↔ Clamping_Shaft_Collar_-_1_2_Hex_ID_217-2737:1
- Mate:441: 30in 1x1 Beam:2 ↔ ARm Gearbox Plate:5
- Mate:442: 30in 1x1 Beam:2 ↔ ARm Gearbox Plate:5
- Mate:443 (76.2 mm): 25in 1x1 Beam:3 ↔ ARm Gearbox Plate:5
- Flush:4: _72t_Aluminum_Plate_Sprocket_25_Chain_1-1_8_Bearing_Bore_217-2627:2 ↔ am-3621 - S25-18HA-500H:1
- Mate:444: Hex Hub:3 ↔ 1_2_Acetal_Spacer_-_1_2_Hex_217-3261:12
- Mate:445: Hex Hub:3 ↔ 1_2_Acetal_Spacer_-_1_2_Hex_217-3261:12
- Mate:446: 0_500_ID_x_1_125_OD_x_0_313_WD_Flanged_Bearing_217-2731:8 ↔ 1_2_Acetal_Spacer_-_1_2_Hex_217-3261:12
- Mate:447: 0_500_ID_x_1_125_OD_x_0_313_WD_Flanged_Bearing_217-2731:8 ↔ 1_2_Acetal_Spacer_-_1_2_Hex_217-3261:12
